# Autodesk Inventor assembly: aim-a-lyzer assy
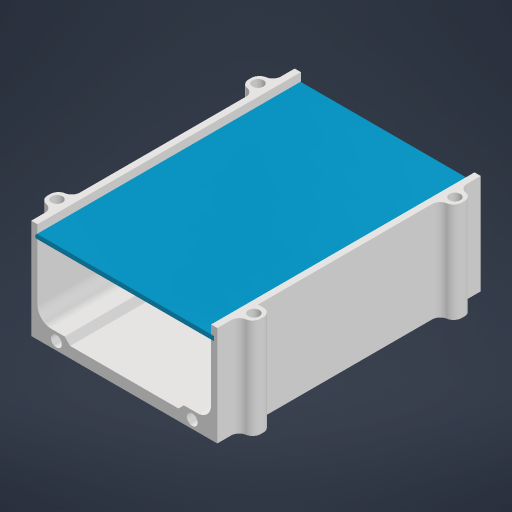
[picture p0: Inventor's stored thumbnail of the model, 512x512]
Saved by Autodesk Inventor 2023 (Build 270158000, 158)
## iProperties
Created: 2024-01-05
Part Number: aim-a-lyzer assy
Document SubType Name: Assembly
Designer: nick_
Author: nick_
## Documents named in this file (3)
- D:\Github\Classpert_GreenTurtles_FinalProject\Mechanical\casing\3dPrintFiles\aim-a-lyzer assy.iam
- D:\Github\Classpert_GreenTurtles_FinalProject\Mechanical\casing\Discovery boar holder.ipt
- D:\Github\Classpert_GreenTurtles_FinalProject\Mechanical\casing\Discovery board.ipt
## Components (2 placed, 2 different names)
1. Discovery boar holder:1 — Mate:1, Flush:1
2. Discovery board:1 — Mate:1, Mate:2, Flush:1
## Relationships (3: Mate 2, Flush 1)
- Mate:1: Discovery boar holder:1 ↔ Discovery board:1
- Mate:2: Discovery board:1
- Flush:1: Discovery boar holder:1 ↔ Discovery board:1
